# Autodesk Inventor assembly: Gear base almost finished
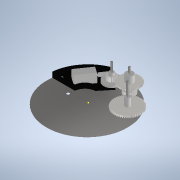
[picture p0: Inventor's stored thumbnail of the model, 180x180]
Saved by Autodesk Inventor 2021 (Build 250183000, 183)
## iProperties
Created: 2020-10-31
Part Number: Gear base almost finished
Document SubType Name: Assembly
Designer: joshualawrence19
Author: joshualawrence19
## Documents named in this file (9)
- H:\design project\Gear base almost finished.iam
- H:\design project\motorbaseplate.ipt
- H:\design project\smallgear.ipt
- H:\design project\thirdgear.ipt
- H:\design project\gearwitspring.ipt
- H:\design project\firstassembly\Design Accelerator\Spur Gears3.iam
- H:\design project\firstassembly\Design Accelerator\Spur Gears4.iam
- H:\design project\motorblack.ipt
- H:\design project\motor.ipt
## Components (8 placed, 7 different names)
1. motorbaseplate:1 — Insert:1, Insert:2, Insert:3, Rotation:2, Insert:4
2. smallgear:1 — Insert:1, Mate:7, Mate:8, Rotation:3
3. thirdgear:1 — Insert:2, Mate:6, Flush:1, Rotation:4
4. gearwitspring:1 — Insert:3, Mate:4, Mate:5, Mate:9, Rotation:2, Rotation:4
5. Spur Gears:2 [sub-assembly] — Mate:4, Mate:5, Mate:6, Flush:1, Mate:10, Rotation:1
6. Spur Gears:3 [sub-assembly] — Mate:7, Mate:8, Mate:9, Mate:10, Rotation:1, Rotation:3
7. motorblack:1 — Insert:4, Mate:11
8. motor:1 — Mate:11
## Relationships (17: Mate 8, Insert 4, RelateRotation 4, Flush 1)
- Insert:1: motorbaseplate:1 ↔ smallgear:1
- Insert:2: motorbaseplate:1 ↔ thirdgear:1
- Insert:3: motorbaseplate:1 ↔ gearwitspring:1
- Mate:4: gearwitspring:1 ↔ Spur Gears:2
- Mate:5: gearwitspring:1 ↔ Spur Gears:2
- Mate:6: thirdgear:1 ↔ Spur Gears:2
- Flush:1: thirdgear:1 ↔ Spur Gears:2
- Mate:7: smallgear:1 ↔ Spur Gears:3
- Mate:8: smallgear:1 ↔ Spur Gears:3
- Mate:9: gearwitspring:1 ↔ Spur Gears:3
- Mate:10: Spur Gears:2 ↔ Spur Gears:3
- Rotation:1 [RelateRotation] (1 ul): Spur Gears:2 ↔ Spur Gears:3
- Rotation:2 [RelateRotation] (3.913 ul): motorbaseplate:1 ↔ gearwitspring:1
- Rotation:3 [RelateRotation] (0.704 ul): smallgear:1 ↔ Spur Gears:3
- Rotation:4 [RelateRotation] (1.484 ul): thirdgear:1 ↔ gearwitspring:1
- Insert:4: motorbaseplate:1 ↔ motorblack:1
- Mate:11: motorblack:1 ↔ motor:1
